# Autodesk Inventor assembly: Servo_Bracket
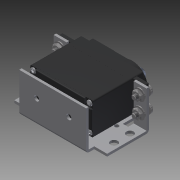
[picture p0: Inventor's stored thumbnail of the model, 180x180]
Saved by Autodesk Inventor 2015 (Build 190159000, 159)
## iProperties
Created: 2015-05-21
Part Number: Servo_Bracket
Document SubType Name: Assembly
Designer: Quinn
Author: Quinn
## Documents named in this file (4)
- C:\Users\Quinn\Desktop\3DCNC Design\InventorModels\Assemblies\FL_Servo_Bracket.iam
- C:\Users\Quinn\Desktop\3DCNC Design\InventorModels\Metal\Brackets\asb-04-ServoMount.ipt
- C:\Users\Quinn\Desktop\3DCNC Design\InventorModels\Electronics\Servo\standard_servo.iam
- C:\Users\Quinn\Desktop\3DCNC Design\InventorModels\Assemblies\FL_Servo_Bracket\Design Accelerator\Bolted Connection1.iam
## Components (7 placed, 3 different names)
1. asb-04-ServoMount:1 — Insert:1, Insert:2, Mate:3, Mate:4
2. standard_servo:1 [sub-assembly] — Insert:1, Mate:1, Mate:2
3. Bolted Connection:1 [sub-assembly] — Mate:1, Mate:2
4. Bolted Connection:2 [sub-assembly]
5. Bolted Connection:3 [sub-assembly] — Insert:2
6. Bolted Connection:4 [sub-assembly] — Mate:4
7. Bolted Connection:5 [sub-assembly] — Mate:3
## Relationships (6: Mate 4, Insert 2)
- Insert:1: asb-04-ServoMount:1 ↔ standard_servo:1
- Mate:1: standard_servo:1 ↔ Bolted Connection:1
- Mate:2: standard_servo:1 ↔ Bolted Connection:1
- Insert:2: asb-04-ServoMount:1 ↔ Bolted Connection:3
- Mate:3: asb-04-ServoMount:1 ↔ Bolted Connection:5
- Mate:4: asb-04-ServoMount:1 ↔ Bolted Connection:4
